# Autodesk Inventor assembly: drawerassem
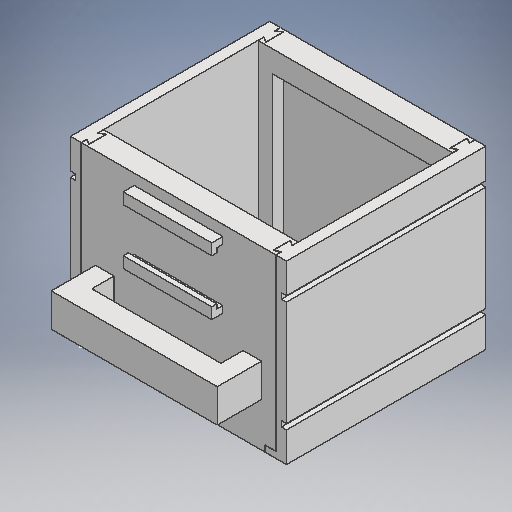
[picture p0: Inventor's stored thumbnail of the model, 512x512]
Saved by Autodesk Inventor 2025.2 (Build 292293000, 293)
## iProperties
Created: 2025-03-25
Part Number: drawerassem
Document SubType Name: Assembly
Designer: Alex
Author: Alex
## Documents named in this file (3)
- C:\Shared\alex-bartella-schoolwork\4b03\dr3\V1\drawerassem.iam
- C:\Shared\alex-bartella-schoolwork\4b03\dr3\V1\drawerside.ipt
- C:\Shared\alex-bartella-schoolwork\4b03\dr3\V1\maindrawer.ipt
## Components (3 placed, 2 different names)
1. drawerside:1 — Mate:1, Mate:2, Mate:3
2. maindrawer:1 — Mate:1, Mate:2, Mate:3, Mate:4, Mate:5, Mate:6
3. drawerside:2 — Mate:4, Mate:5, Mate:6
## Relationships (6: Mate 6)
- Mate:1 (0.1 mm): drawerside:1 ↔ maindrawer:1
- Mate:2 (0.1 mm): drawerside:1 ↔ maindrawer:1
- Mate:3 (0.1 mm): drawerside:1 ↔ maindrawer:1
- Mate:4 (0.1 mm): maindrawer:1 ↔ drawerside:2
- Mate:5 (0.1 mm): maindrawer:1 ↔ drawerside:2
- Mate:6 (0.1 mm): maindrawer:1 ↔ drawerside:2
## Named parameters: tol = 0.1 mm
